# Autodesk Inventor assembly: Mitutoyo-BD-Plan-Apo-system
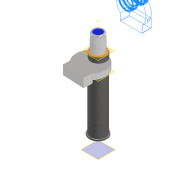
[picture p0: Inventor's stored thumbnail of the model, 180x180]
Saved by Autodesk Inventor 2021 (Build 250183000, 183)
## iProperties
Created: 2022-09-08
Part Number: Mitutoyo-BD-Plan-Apo-system
Document SubType Name: Assembly
Designer: Nikita
Author: Nikita
## Documents named in this file (7)
- C:\Users\Public\GitHub-public\benchtop-hardware\Benchtop\CAD-model-Inventor2021\mesoSPIM\detection_path\Mitutoyo\Mitutoyo-BD-Plan-Apo-system.iam
- C:\Users\Public\GitHub-public\benchtop-hardware\Benchtop\CAD-model-Inventor2021\library\Mitutoyo\BD-Plan-Apo-approx.ipt
- C:\Users\Public\GitHub-public\benchtop-hardware\Benchtop\CAD-model-Inventor2021\library\Thorlabs\accessoires\M2M40S.ipt
- C:\Users\Public\GitHub-public\benchtop-hardware\Benchtop\CAD-model-Inventor2021\library\Thorlabs\lens_tubes\SM2E60.ipt
- C:\Users\Public\GitHub-public\benchtop-hardware\Benchtop\CAD-model-Inventor2021\library\Thorlabs\f-mounts\SM2NFM2.ipt
- C:\Users\Public\GitHub-public\benchtop-hardware\Benchtop\CAD-model-Inventor2021\library\Thorlabs\lens_tubes\SM2M20.ipt
- C:\Users\Public\GitHub-public\benchtop-hardware\Benchtop\CAD-model-Inventor2021\library\ZWO-EWF(filter_wheel)\ZWO-EFWMini+SM2-adapters.iam
## Components (6 placed, 6 different names)
1. Mitutoyo-BD-Plan-Apo-approx:1 — Insert:1
2. M2M40S:Adapter — Insert:1, Flush:2, Insert:6
3. SM2E60:L=150mm — Flush:1, Insert:4, Mate:1, Insert:5
4. SM2NFM2:3 — Insert:4
5. SM2M20:1 — Mate:1
6. ZWO-EFWMini+SM2-adapters:1 [sub-assembly] — Insert:5, Insert:6
## Relationships (7: Insert 4, Flush 2, Mate 1)
- Insert:1: Mitutoyo-BD-Plan-Apo-approx:1 ↔ M2M40S:Adapter
- Flush:1 (-10 mm): SM2E60:L=150mm
- Flush:2: M2M40S:Adapter
- Insert:4 (-210 mm): SM2E60:L=150mm ↔ SM2NFM2:3
- Mate:1: SM2E60:L=150mm ↔ SM2M20:1
- Insert:5: SM2E60:L=150mm ↔ ZWO-EFWMini+SM2-adapters:1
- Insert:6: M2M40S:Adapter ↔ ZWO-EFWMini+SM2-adapters:1
